# Autodesk Inventor assembly: Assembly9
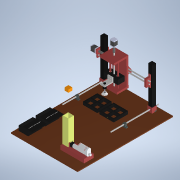
[picture p0: Inventor's stored thumbnail of the model, 180x180]
Saved by Autodesk Inventor 2021 (Build 250183000, 183)
## iProperties
Created: 2023-10-30
Part Number: Assembly9
Document SubType Name: Assembly
Designer: habib
Author: habib
## Documents named in this file (7)
- C:\Users\habib\Desktop\MATfinalisa\Assembly9.iam
- C:\Users\habib\Desktop\design1_project\lastnew\tableiso.ipt
- C:\Users\habib\Desktop\design1_project\lastnew\cartisolated.ipt
- C:\Users\habib\Desktop\design1_project\lastnew\cuboid.ipt
- C:\Users\habib\Desktop\design1_project\lastnew\feedingpressisolated.ipt
- C:\Users\habib\Desktop\design1_project\lastnew\gripperrrisolated.ipt
- C:\Users\habib\Desktop\design1_project\lastnew\CARTESIAAAN.ipt
## Components (6 placed, 6 different names)
1. tableiso:1 — Mate:1, Mate:2, Mate:5
2. cartisolated:1 — Mate:3, Mate:4
3. cuboid:1
4. feedingpressisolated:1 — Mate:5
5. gripperrrisolated:1 — Mate:4
6. CARTESIAAAN:1 — Mate:1, Mate:2, Mate:3
## Relationships (5: Mate 5)
- Mate:1: tableiso:1 ↔ CARTESIAAAN:1
- Mate:2: tableiso:1 ↔ CARTESIAAAN:1
- Mate:3: cartisolated:1 ↔ CARTESIAAAN:1
- Mate:4: cartisolated:1 ↔ gripperrrisolated:1
- Mate:5: tableiso:1 ↔ feedingpressisolated:1
